# Autodesk Inventor assembly: Subassembly1
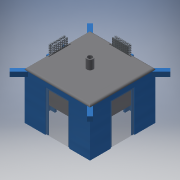
[picture p0: Inventor's stored thumbnail of the model, 180x180]
Saved by Autodesk Inventor 2017 (Build 210142000, 142)
## iProperties
Created: 2017-01-05
Part Number: Subassembly1
Document SubType Name: Assembly
Designer: jbui8
Author: jbui8
## Documents named in this file (7)
- C:\Users\jbui8\Dropbox\CAD Designs for Research and Work\PV Electrolyzer\Reactor Design\Reactor Parts\Assembly Parts\Subassembly1.iam
- C:\Users\jbui8\Dropbox\CAD Designs for Research and Work\PV Electrolyzer\Reactor Design\Reactor Parts\Assembly Parts\Reactor Main Body.ipt
- C:\Users\jbui8\Dropbox\CAD Designs for Research and Work\PV Electrolyzer\Reactor Design\Reactor Parts\Assembly Parts\Reactor Lid.ipt
- C:\Users\jbui8\Dropbox\CAD Designs for Research and Work\PV Electrolyzer\Reactor Design\Reactor Parts\Assembly Parts\Reactor Glass.ipt
- C:\Users\jbui8\Dropbox\CAD Designs for Research and Work\PV Electrolyzer\Reactor Design\Reactor Parts\Assembly Parts\Reactor Meshes.ipt
- C:\Users\jbui8\Dropbox\CAD Designs for Research and Work\PV Electrolyzer\Reactor Design\Reactor Parts\Assembly Parts\Reactor Meshes_MIR.ipt
- C:\Users\jbui8\Dropbox\CAD Designs for Research and Work\PV Electrolyzer\Reactor Design\Reactor Parts\Assembly Parts\Reactor Meshes_MIR1.ipt
## Components (8 placed, 6 different names)
1. Reactor Main Body:1 — Mate:1, Mate:2, Mate:3, Mate:4, Mate:14, Mate:15, Mate:16, Mate:17, Mate:19, Mate:21, Symmetry:2
2. Reactor Lid:1 — Mate:2, Mate:3, Mate:4, Mate:18, Mate:20, Symmetry:1
3. Reactor Glass:1 — Mate:14, Mate:15
4. Reactor Glass:2 — Mate:16, Mate:17
5. Reactor Meshes:1 — Mate:18, Mate:19, Symmetry:2
6. Reactor Meshes:2 — Mate:20, Mate:21, Symmetry:1
7. Reactor Meshes_MIR:1
8. Reactor Meshes_MIR1:1
## Relationships (14: Mate 12, Symmetry 2)
- Mate:1: Reactor Main Body:1
- Mate:2 (1 mm): Reactor Main Body:1 ↔ Reactor Lid:1
- Mate:3 (1 mm): Reactor Main Body:1 ↔ Reactor Lid:1
- Mate:4: Reactor Main Body:1 ↔ Reactor Lid:1
- Mate:14: Reactor Main Body:1 ↔ Reactor Glass:1
- Mate:15: Reactor Main Body:1 ↔ Reactor Glass:1
- Mate:16: Reactor Main Body:1 ↔ Reactor Glass:2
- Mate:17: Reactor Main Body:1 ↔ Reactor Glass:2
- Mate:18: Reactor Lid:1 ↔ Reactor Meshes:1
- Mate:19: Reactor Main Body:1 ↔ Reactor Meshes:1
- Mate:20: Reactor Lid:1 ↔ Reactor Meshes:2
- Mate:21: Reactor Main Body:1 ↔ Reactor Meshes:2
- Symmetry:1: Reactor Lid:1 ↔ Reactor Meshes:2
- Symmetry:2: Reactor Main Body:1 ↔ Reactor Meshes:1
